# Autodesk Inventor assembly: Vertical Lift
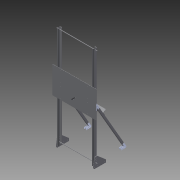
[picture p0: Inventor's stored thumbnail of the model, 180x180]
Saved by Autodesk Inventor 2015 SP1 (Build 190203100, 203)
## iProperties
Created: 2015-01-13
Part Number: Vertical Lift
Document SubType Name: Assembly
Designer: Jarod
Author: Jarod
## Documents named in this file (15)
- C:\Users\Jarod\Documents\Westview\Robotics\FRC\2015\CAD\Robot\Vertical Lift\Vertical Lift.iam
- C:\Users\Jarod\Documents\Westview\Robotics\FRC\2015\CAD\Robot\Vertical Lift\garage door 2in rail.ipt
- C:\Users\Jarod\Documents\Westview\Robotics\FRC\2015\CAD\Robot\Vertical Lift\garage door 2in roller.ipt
- C:\Users\Jarod\Documents\Westview\Robotics\FRC\2015\CAD\Robot\Vertical Lift\garage door hinge.ipt
- C:\Users\Jarod\Documents\Westview\Robotics\FRC\2015\CAD\Robot\Vertical Lift\lift plate.ipt
- C:\Users\Jarod\Documents\Westview\Robotics\FRC\2015\CAD\Robot\Vertical Lift\Imported Components\VEXpro-VersaPlanetary-2stage-with-BAG\VEXpro-VersaPlanetary-2stage-with-BAG.iam
- C:\Users\Jarod\Documents\Westview\Robotics\FRC\2015\CAD\Robot\Vertical Lift\rail aligner.ipt
- C:\Users\Jarod\Documents\Westview\Robotics\FRC\2015\CAD\Robot\Vertical Lift\garage door 2in rail_MIR.ipt
- C:\Users\Jarod\Documents\Westview\Robotics\FRC\2015\CAD\Robot\Vertical Lift\rail mounting bracket.ipt
- C:\Users\Jarod\Documents\Westview\Robotics\FRC\2015\CAD\Robot\Vertical Lift\0.375 axle.ipt
- C:\Users\Jarod\Documents\Westview\Robotics\FRC\2015\CAD\Robot\Vertical Lift\Imported Components\0.375 shaft collar\0.375 shaft collar.ipt
- C:\Users\Jarod\Documents\Westview\Robotics\FRC\2015\CAD\Robot\Vertical Lift\Imported Components\Versaframe 30deg gusset\Versaframe 30deg gusset.ipt
- C:\Users\Jarod\Documents\Westview\Robotics\FRC\2015\CAD\Robot\Vertical Lift\Imported Components\Versaframe 60deg gusset\Versaframe 60deg gusset.ipt
- C:\Users\Jarod\Documents\Westview\Robotics\FRC\2015\CAD\Robot\Vertical Lift\1x1 support.ipt
- C:\Users\Jarod\Documents\Westview\Robotics\FRC\2015\CAD\Robot\Vertical Lift\2x2 angle support.ipt
## Components (33 placed, 14 different names)
1. garage door 2in rail:1 — Mate:4, Mate:5, Mate:44, Flush:5, Mate:45, Flush:7, Mate:48, Flush:8, Mate:90, Mate:91, Mate:94, Mate:108, Mate:110, Mate:111, Mate:112, Flush:20
2. garage door 2in rail_MIR:1 — Mate:46, Mate:47, Flush:6, Flush:7, Mate:48, Mate:49, Mate:50, Mate:92, Flush:9, Mate:93, Mate:95, Mate:96, Flush:11, Mate:98, Mate:104, Mate:106, Mate:113, Mate:114, Flush:21
3. garage door 2in roller:1 — Mate:10, Mate:12, Mate:94
4. garage door 2in roller:2 — Mate:4, Mate:5, Mate:11, Mate:13
5. garage door 2in roller:3 — Mate:10, Mate:14, Mate:50, Mate:95
6. garage door 2in roller:4 — Mate:11, Mate:15, Mate:49, Mate:96
7. garage door hinge:1 — Mate:12, Mate:20, Mate:21
8. garage door hinge:2 — Mate:13, Mate:23, Mate:25
9. garage door hinge:3 — Mate:14, Mate:22
10. garage door hinge:4 — Mate:15, Mate:24
11. lift plate:1 — Mate:20, Mate:21, Mate:22, Mate:23, Mate:24, Mate:25, Mate:26, Mate:27, Mate:28
12. VEXpro-VersaPlanetary-2stage-with-BAG:1 [sub-assembly] — Mate:26, Mate:27, Mate:28
13. rail aligner:1 — Mate:46, Mate:47, Flush:6
14. rail aligner:2 — Mate:44, Flush:5, Mate:45
15. rail mounting bracket:1 — Flush:8, Mate:90, Mate:91, Mate:102
16. rail mounting bracket:2 — Mate:92, Flush:9, Mate:93, Mate:97, Flush:10, Mate:100
17. 0.375 axle:1 — Mate:97, Flush:10, Mate:99, Mate:101
18. 0.375 axle:2 — Flush:11, Mate:98, Mate:103, Mate:105, Mate:107, Mate:109
19. 0.375 shaft collar:1 — Mate:99, Mate:100
20. 0.375 shaft collar:2 — Mate:101, Mate:102
21. 0.375 shaft collar:3 — Mate:103, Mate:104
22. 0.375 shaft collar:4 — Mate:105, Mate:106
23. 0.375 shaft collar:5 — Mate:107, Mate:108
24. 0.375 shaft collar:6 — Mate:109, Mate:110
25. Versaframe 30deg gusset:1 — Mate:111, Mate:112, Mate:115, Flush:12, Mate:124, Mate:130
26. Versaframe 30deg gusset:2 — Mate:113, Mate:114, Mate:116, Flush:13, Mate:127, Mate:131
27. Versaframe 60deg gusset:1 — Mate:117, Flush:14, Flush:18, Flush:20, Mate:121, Mate:122
28. Versaframe 60deg gusset:2 — Mate:118, Flush:15, Flush:18
29. Versaframe 60deg gusset:3 — Mate:119, Flush:16, Flush:19, Mate:125, Mate:126
30. Versaframe 60deg gusset:4 — Mate:120, Flush:17, Flush:19, Flush:21
31. 1x1 support:1 — Mate:115, Flush:12, Mate:117, Flush:14, Mate:118, Flush:15, Mate:121, Mate:122, Mate:124, Mate:129, Flush:22, Flush:23, Mate:130
32. 1x1 support:2 — Mate:116, Flush:13, Mate:119, Flush:16, Mate:120, Flush:17, Mate:125, Mate:126, Mate:127, Mate:131
33. 2x2 angle support:1 — Mate:129, Flush:22, Flush:23
## Relationships (83: Mate 64, Flush 19)
- Mate:4 (6.35 mm): garage door 2in rail:1 ↔ garage door 2in roller:2
- Mate:5 (28.575 mm): garage door 2in rail:1 ↔ garage door 2in roller:2
- Mate:10: garage door 2in roller:1 ↔ garage door 2in roller:3
- Mate:11: garage door 2in roller:2 ↔ garage door 2in roller:4
- Mate:12: garage door 2in roller:1 ↔ garage door hinge:1
- Mate:13: garage door 2in roller:2 ↔ garage door hinge:2
- Mate:14: garage door 2in roller:3 ↔ garage door hinge:3
- Mate:15: garage door 2in roller:4 ↔ garage door hinge:4
- Mate:20: garage door hinge:1 ↔ lift plate:1
- Mate:21: garage door hinge:1 ↔ lift plate:1
- Mate:22: garage door hinge:3 ↔ lift plate:1
- Mate:23: garage door hinge:2 ↔ lift plate:1
- Mate:24: garage door hinge:4 ↔ lift plate:1
- Mate:25: garage door hinge:2 ↔ lift plate:1
- Mate:26: lift plate:1 ↔ VEXpro-VersaPlanetary-2stage-with-BAG:1
- Mate:27: lift plate:1 ↔ VEXpro-VersaPlanetary-2stage-with-BAG:1
- Mate:28: lift plate:1 ↔ VEXpro-VersaPlanetary-2stage-with-BAG:1
- Mate:44: garage door 2in rail:1 ↔ rail aligner:2
- Flush:5: garage door 2in rail:1 ↔ rail aligner:2
- Mate:45: garage door 2in rail:1 ↔ rail aligner:2
- Mate:46: garage door 2in rail_MIR:1 ↔ rail aligner:1
- Mate:47: garage door 2in rail_MIR:1 ↔ rail aligner:1
- Flush:6: garage door 2in rail_MIR:1 ↔ rail aligner:1
- Flush:7: garage door 2in rail:1 ↔ garage door 2in rail_MIR:1
- Mate:48 (-552.45 mm): garage door 2in rail:1 ↔ garage door 2in rail_MIR:1
- Mate:49 (28.575 mm): garage door 2in rail_MIR:1 ↔ garage door 2in roller:4
- Mate:50 (28.575 mm): garage door 2in rail_MIR:1 ↔ garage door 2in roller:3
- Flush:8 (-38.1 mm): garage door 2in rail:1 ↔ rail mounting bracket:1
- Mate:90: garage door 2in rail:1 ↔ rail mounting bracket:1
- Mate:91: garage door 2in rail:1 ↔ rail mounting bracket:1
- Mate:92: garage door 2in rail_MIR:1 ↔ rail mounting bracket:2
- Flush:9 (-38.1 mm): garage door 2in rail_MIR:1 ↔ rail mounting bracket:2
- Mate:93: garage door 2in rail_MIR:1 ↔ rail mounting bracket:2
- Mate:94 (6.35 mm): garage door 2in rail:1 ↔ garage door 2in roller:1
- Mate:95 (6.35 mm): garage door 2in rail_MIR:1 ↔ garage door 2in roller:3
- Mate:96 (6.35 mm): garage door 2in rail_MIR:1 ↔ garage door 2in roller:4
- Mate:97: rail mounting bracket:2 ↔ 0.375 axle:1
- Flush:10 (-22.225 mm): rail mounting bracket:2 ↔ 0.375 axle:1
- Flush:11 (-28.575 mm): garage door 2in rail_MIR:1 ↔ 0.375 axle:2
- Mate:98: garage door 2in rail_MIR:1 ↔ 0.375 axle:2
- Mate:99: 0.375 axle:1 ↔ 0.375 shaft collar:1
- Mate:100: rail mounting bracket:2 ↔ 0.375 shaft collar:1
- Mate:101: 0.375 axle:1 ↔ 0.375 shaft collar:2
- Mate:102: rail mounting bracket:1 ↔ 0.375 shaft collar:2
- Mate:103: 0.375 axle:2 ↔ 0.375 shaft collar:3
- Mate:104: garage door 2in rail_MIR:1 ↔ 0.375 shaft collar:3
- Mate:105: 0.375 axle:2 ↔ 0.375 shaft collar:4
- Mate:106: garage door 2in rail_MIR:1 ↔ 0.375 shaft collar:4
- Mate:107: 0.375 axle:2 ↔ 0.375 shaft collar:5
- Mate:108: garage door 2in rail:1 ↔ 0.375 shaft collar:5
- Mate:109: 0.375 axle:2 ↔ 0.375 shaft collar:6
- Mate:110: garage door 2in rail:1 ↔ 0.375 shaft collar:6
- Mate:111 (-25.4 mm): garage door 2in rail:1 ↔ Versaframe 30deg gusset:1
- Mate:112: garage door 2in rail:1 ↔ Versaframe 30deg gusset:1
- Mate:113: garage door 2in rail_MIR:1 ↔ Versaframe 30deg gusset:2
- Mate:114 (-25.4 mm): garage door 2in rail_MIR:1 ↔ Versaframe 30deg gusset:2
- Mate:115: Versaframe 30deg gusset:1 ↔ 1x1 support:1
- Flush:12: Versaframe 30deg gusset:1 ↔ 1x1 support:1
- Mate:116: Versaframe 30deg gusset:2 ↔ 1x1 support:2
- Flush:13: Versaframe 30deg gusset:2 ↔ 1x1 support:2
- Mate:117: Versaframe 60deg gusset:1 ↔ 1x1 support:1
- Flush:14: Versaframe 60deg gusset:1 ↔ 1x1 support:1
- Mate:118: Versaframe 60deg gusset:2 ↔ 1x1 support:1
- Flush:15: Versaframe 60deg gusset:2 ↔ 1x1 support:1
- Mate:119: Versaframe 60deg gusset:3 ↔ 1x1 support:2
- Flush:16: Versaframe 60deg gusset:3 ↔ 1x1 support:2
- Mate:120: Versaframe 60deg gusset:4 ↔ 1x1 support:2
- Flush:17: Versaframe 60deg gusset:4 ↔ 1x1 support:2
- Flush:18: Versaframe 60deg gusset:1 ↔ Versaframe 60deg gusset:2
- Flush:19: Versaframe 60deg gusset:3 ↔ Versaframe 60deg gusset:4
- Flush:20: garage door 2in rail:1 ↔ Versaframe 60deg gusset:1
- Flush:21: garage door 2in rail_MIR:1 ↔ Versaframe 60deg gusset:4
- Mate:121 (0.127 mm): Versaframe 60deg gusset:1 ↔ 1x1 support:1
- Mate:122 (0.127 mm): Versaframe 60deg gusset:1 ↔ 1x1 support:1
- Mate:124 (0.127 mm): Versaframe 30deg gusset:1 ↔ 1x1 support:1
- Mate:125 (0.127 mm): Versaframe 60deg gusset:3 ↔ 1x1 support:2
- Mate:126 (0.127 mm): Versaframe 60deg gusset:3 ↔ 1x1 support:2
- Mate:127 (0.127 mm): Versaframe 30deg gusset:2 ↔ 1x1 support:2
- Mate:129: 1x1 support:1 ↔ 2x2 angle support:1
- Flush:22: 1x1 support:1 ↔ 2x2 angle support:1
- Flush:23 (622.3 mm): 1x1 support:1 ↔ 2x2 angle support:1
- Mate:130 (0.127 mm): Versaframe 30deg gusset:1 ↔ 1x1 support:1
- Mate:131 (0.127 mm): Versaframe 30deg gusset:2 ↔ 1x1 support:2
